# Autodesk Inventor assembly: ЛЦМК000002.00.05.00.02.00 2 xiao
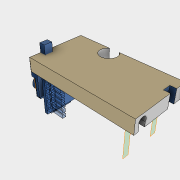
[picture p0: Inventor's stored thumbnail of the model, 180x180]
Saved by Autodesk Inventor 2021.2 (Build 252289000, 289)
## iProperties
Created: 2025-11-21
Part Number: ЛЦМК000002.00.05.00.02.00 2 xiao
Document SubType Name: Assembly
Designer: Захаров
Author: Захаров
## Documents named in this file (3)
- C:\Users\User\Documents\CaseARHead1\ЛЦМК000002.00.05.00.02.00 2 xiao.iam
- C:\Users\User\Documents\CaseARHead1\ЛЦМК.00002.00.00.00.00.22-01 Компактный короб.ipt
- C:\Users\User\Documents\CaseARHead1\Сборка1.iam
## Components (2 placed, 2 different names)
1. ЛЦМК.00002.00.00.00.00.22-01 Компактный короб:1 — Заподлицо:1, Совмещение:1, Заподлицо:2
2. Сборка1:1 [sub-assembly] — Заподлицо:1, Совмещение:1, Заподлицо:2
## Relationships (3: Flush 2, Mate 1)
- Заподлицо:1 [Flush]: ЛЦМК.00002.00.00.00.00.22-01 Компактный короб:1 ↔ Сборка1:1
- Совмещение:1 [Mate] (-2 mm): ЛЦМК.00002.00.00.00.00.22-01 Компактный короб:1 ↔ Сборка1:1
- Заподлицо:2 [Flush] (2.5 mm): ЛЦМК.00002.00.00.00.00.22-01 Компактный короб:1 ↔ Сборка1:1
